# Autodesk Inventor assembly: Assembly1
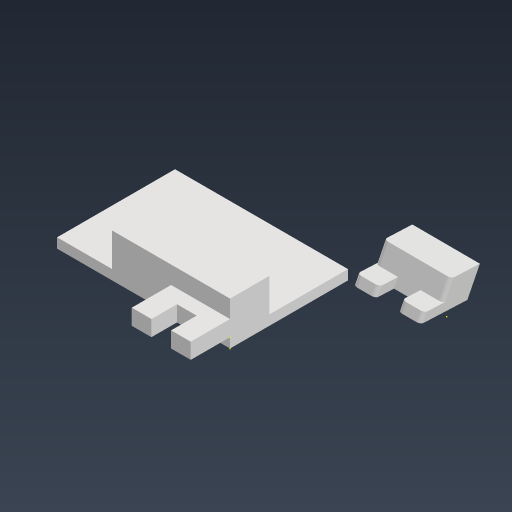
[picture p0: Inventor's stored thumbnail of the model, 512x512]
Saved by Autodesk Inventor 2024 (Build 280153000, 153)
## iProperties
Created: 2023-12-26
Part Number: Assembly1
Document SubType Name: Assembly
Designer: Piter
Author: Piter
## Documents named in this file (4)
- C:\Users\Piter\OneDrive\Pulpit\Modele\My-3D-printing-projects\Assembly1.iam
- C:\Users\Piter\OneDrive\Pulpit\Modele\My-3D-printing-projects\millenium_back_R.ipt
- C:\Users\Piter\OneDrive\Pulpit\Modele\My-3D-printing-projects\sklejka.ipt
- C:\Users\Piter\OneDrive\Pulpit\Modele\My-3D-printing-projects\millenium.ipt
## Components (3 placed, 3 different names)
1. millenium_back_R:1
2. sklejka:1 — Flush:1, Mate:1, Mate:2
3. millenium:1 — Flush:1, Mate:1, Mate:2
## Relationships (3: Mate 2, Flush 1)
- Flush:1: sklejka:1 ↔ millenium:1
- Mate:1: sklejka:1 ↔ millenium:1
- Mate:2: sklejka:1 ↔ millenium:1
